# Autodesk Inventor assembly: Controller_Asem
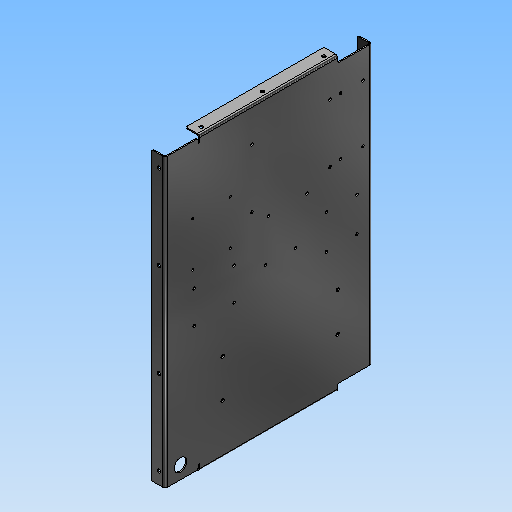
[picture p0: Inventor's stored thumbnail of the model, 512x512]
Saved by Autodesk Inventor 2020 (Build 240168000, 168)
## iProperties
Created: 2021-05-11
Part Number: Controller_Asem
Document SubType Name: Assembly
Designer: ken113
Author: ken113
## Documents named in this file (7)
- C:\Users\lvglv\Documents\GitHub\Cheap_Belt_Printer\Model\Asem\Controller_Asem.iam
- C:\Users\lvglv\Documents\GitHub\Cheap_Belt_Printer\Model\Parts\Electrical_Components\mean-well-lrs-350-24-1.snapshot.3\meanwell_lrs-350-24_UPDATED.ipt
- C:\Users\lvglv\Documents\GitHub\Cheap_Belt_Printer\Model\Parts\Electrical_Components\biqu-heat-bed-power-module-expansion-hot-bed-mos-tube-for-3d-printer-1.snapshot.2\BIQU-3D0109.iam
- C:\Users\lvglv\Documents\GitHub\Cheap_Belt_Printer\Model\Parts\Electrical_Components\BIGTREETECH_SKR_V1.4\BTT_SKR_V1.4 v13_TOP.iam
- C:\Users\lvglv\Documents\GitHub\Cheap_Belt_Printer\Model\Parts\Meviy\Board_Mount.ipt
- C:\Users\lvglv\Documents\GitHub\Cheap_Belt_Printer\Model\Parts\Grabcad\raspberry-pi-4-model-b-03-1.snapshot.1\Raspberry-Pi-4-Model-B-03.ipt
- C:\Users\lvglv\Documents\GitHub\Cheap_Belt_Printer\Model\Parts\Grabcad\psu-meanwell-5vdc-15watts-1.snapshot.1\Mean Well RS-15-5.ipt
## Components (6 placed, 6 different names)
1. meanwell_lrs-350-24_UPDATED:1 — 挿入:1, 挿入:2
2. BIQU-3D0109:1 [sub-assembly] — 挿入:5, メイト:1
3. BTT_SKR_V1.4 v13_TOP:1 [sub-assembly] — 挿入:3, 挿入:4
4. Board_Mount:1 — 挿入:1, 挿入:2, 挿入:3, 挿入:4, 挿入:5, メイト:1, メイト:2, 角度:1, メイト:3, 挿入:6
5. Raspberry-Pi-4-Model-B-03:1 — メイト:2, 角度:1, メイト:3
6. Mean Well RS-15-5:1 — 挿入:6
## Relationships (10: Insert 6, Mate 3, Angle 1)
- 挿入:1 [Insert]: meanwell_lrs-350-24_UPDATED:1 ↔ Board_Mount:1
- 挿入:2 [Insert]: meanwell_lrs-350-24_UPDATED:1 ↔ Board_Mount:1
- 挿入:3 [Insert] (5 mm): BTT_SKR_V1.4 v13_TOP:1 ↔ Board_Mount:1
- 挿入:4 [Insert] (5 mm): BTT_SKR_V1.4 v13_TOP:1 ↔ Board_Mount:1
- 挿入:5 [Insert] (5 mm): BIQU-3D0109:1 ↔ Board_Mount:1
- メイト:1 [Mate]: BIQU-3D0109:1 ↔ Board_Mount:1
- メイト:2 [Mate] (5 mm): Board_Mount:1 ↔ Raspberry-Pi-4-Model-B-03:1
- 角度:1 [Angle] (180 deg): Board_Mount:1 ↔ Raspberry-Pi-4-Model-B-03:1
- メイト:3 [Mate]: Board_Mount:1 ↔ Raspberry-Pi-4-Model-B-03:1
- 挿入:6 [Insert]: Board_Mount:1 ↔ Mean Well RS-15-5:1
